# Autodesk Inventor assembly: fab model mk-1
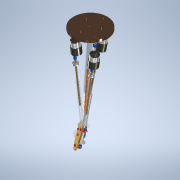
[picture p0: Inventor's stored thumbnail of the model, 180x180]
Saved by Autodesk Inventor 2020 (Build 240168000, 168)
## iProperties
Created: 2020-12-19
Part Number: fab model mk-1
Document SubType Name: Assembly
Designer: Vikki
Author: Vikki
## Documents named in this file (16)
- D:\borewell rescuebot\pll manipulator files\sps manipulator\fab model mk-1.iam
- D:\borewell rescuebot\pll manipulator files\sps manipulator\base.ipt
- D:\borewell rescuebot\pll manipulator files\sps manipulator\craftsman-3-pc-universal-joint-set-1.snapshot.1\Craftsman Socket U-Joint.iam
- D:\borewell rescuebot\pll manipulator files\sps manipulator\platform.ipt
- D:\borewell rescuebot\pll manipulator files\sps manipulator\JGB37-520.iam
- D:\borewell rescuebot\pll manipulator files\sps manipulator\leadscrew.ipt
- D:\borewell rescuebot\pll manipulator files\sps manipulator\coupler.ipt
- D:\borewell rescuebot\pll manipulator files\sps manipulator\telescopic boom1.ipt
- D:\borewell rescuebot\pll manipulator files\sps manipulator\boom 3.ipt
- D:\borewell rescuebot\pll manipulator files\sps manipulator\15.ipt
- D:\borewell rescuebot\pll manipulator files\sps manipulator\ball-pin.ipt
- D:\borewell rescuebot\2020 bot\borewell max sixe.ipt
- D:\borewell rescuebot\2020 bot\min size bore well.ipt
- D:\borewell rescuebot\pll manipulator files\sps manipulator\motor bracket.ipt
- D:\borewell rescuebot\pll manipulator files\sps manipulator\fab model mk-1\Design Accelerator\Bearing1.iam
- D:\borewell rescuebot\pll manipulator files\sps manipulator\connector plunger.ipt
## Components (39 placed, 15 different names)
1. base:1 — Mate:1, Mate:2, Mate:3, Mate:4, Mate:5, Mate:6, Angle:1, Mate:18, Mate:19, Flush:2, Angle:7, Mate:61, Flush:6
2. Craftsman Socket U-Joint:1 [sub-assembly] — Mate:1, Mate:2, Angle:2, Mate:25, Mate:34, Mate:35, Angle:9, Mate:69
3. Craftsman Socket U-Joint:2 [sub-assembly] — Mate:5, Mate:6, Angle:3, Mate:24, Mate:32, Mate:33, Angle:10, Mate:75
4. Craftsman Socket U-Joint:3 [sub-assembly] — Mate:3, Mate:4, Angle:1, Angle:2, Angle:3, Mate:23, Mate:29, Mate:30, Angle:8, Mate:72
5. platform:1 — Mate:7, Mate:8, Mate:9, Mate:10, Mate:11, Mate:12, Mate:16, Mate:17, Flush:2, Angle:6, Angle:7, Mate:63, Flush:8, Mate:64, Mate:65, Flush:9, Flush:10
6. Craftsman Socket U-Joint:4 [sub-assembly] — Mate:7, Mate:8, Mate:24, Mate:55, Mate:82, Mate:85
7. Craftsman Socket U-Joint:5 [sub-assembly] — Mate:9, Mate:12, Mate:25, Mate:53, Mate:86, Mate:88
8. Craftsman Socket U-Joint:6 [sub-assembly] — Mate:10, Mate:11, Mate:23, Mate:57, Mate:78, Mate:81
9. Craftsman Socket U-Joint:7 [sub-assembly] — Mate:16, Mate:17, Mate:26, Flush:1, Angle:6, Mate:52, Mate:60
10. Craftsman Socket U-Joint:8 [sub-assembly] — Mate:18, Mate:19, Angle:5, Mate:26, Flush:1, Mate:48, Mate:59
11. JGB37-520:1 [sub-assembly] — Mate:29, Mate:30, Angle:8, Mate:43, Mate:47, Mate:73, Mate:74
12. JGB37-520:2 [sub-assembly] — Mate:32, Mate:33, Angle:10, Mate:44, Mate:46, Mate:76, Mate:77
13. JGB37-520:3 [sub-assembly] — Mate:34, Mate:35, Angle:9, Mate:36, Mate:45, Flush:7, Mate:70
14. leadscrew:1 — Mate:36, Mate:37, Mate:38
15. coupler:1 — Mate:37, Mate:38, Mate:45, Mate:67
16. leadscrew:2
17. coupler:2 — Mate:43, Mate:47
18. leadscrew:3
19. coupler:3 — Mate:44, Mate:46
20. telescopic boom1:1 — Mate:48, Mate:51, Mate:59
21. boom 3:1 — Mate:51, Mate:52
22. 15:1 — Mate:53, Angle:13, Mate:87
23. 15:2 — Mate:57, Angle:12, Mate:79, Mate:80
24. 15:3 — Mate:55, Angle:11, Mate:83, Mate:84
25. ball-pin:1 — Mate:60
26. borewell max sixe:1 — Mate:61, Mate:62, Flush:5
27. min size bore well:1 — Mate:62, Flush:5, Flush:6
28. motor bracket:1 — Flush:7, Mate:66, Mate:69, Mate:70, Angle:13
29. Bearing:1 [sub-assembly] — Mate:63, Flush:8
30. Bearing:2 [sub-assembly] — Mate:64, Flush:10
31. Bearing:3 [sub-assembly] — Mate:65, Flush:9
32. Bearing:4 [sub-assembly] — Mate:66, Mate:67
33. motor bracket:2 — Flush:11, Mate:72, Mate:73, Mate:74, Angle:12
34. Bearing:5 [sub-assembly] — Flush:11
35. motor bracket:3 — Mate:75, Mate:76, Mate:77, Angle:11
36. Bearing:6 [sub-assembly]
37. connector plunger:1 — Mate:78, Mate:79, Mate:80, Mate:81
38. connector plunger:2 — Mate:86, Mate:87, Mate:88
39. connector plunger:3 — Mate:82, Mate:83, Mate:84, Mate:85
## Relationships (98: Mate 74, Angle 12, Flush 12)
- Mate:1: base:1 ↔ Craftsman Socket U-Joint:1
- Mate:2: base:1 ↔ Craftsman Socket U-Joint:1
- Mate:3: base:1 ↔ Craftsman Socket U-Joint:3
- Mate:4: base:1 ↔ Craftsman Socket U-Joint:3
- Mate:5: base:1 ↔ Craftsman Socket U-Joint:2
- Mate:6: base:1 ↔ Craftsman Socket U-Joint:2
- Mate:7: platform:1 ↔ Craftsman Socket U-Joint:4
- Mate:8: platform:1 ↔ Craftsman Socket U-Joint:4
- Mate:9: platform:1 ↔ Craftsman Socket U-Joint:5
- Mate:10: platform:1 ↔ Craftsman Socket U-Joint:6
- Mate:11: platform:1 ↔ Craftsman Socket U-Joint:6
- Mate:12: platform:1 ↔ Craftsman Socket U-Joint:5
- Angle:1 (30 deg): base:1 ↔ Craftsman Socket U-Joint:3
- Angle:2 (60 deg): Craftsman Socket U-Joint:1 ↔ Craftsman Socket U-Joint:3
- Angle:3 (120 deg): Craftsman Socket U-Joint:2 ↔ Craftsman Socket U-Joint:3
- Mate:16: platform:1 ↔ Craftsman Socket U-Joint:7
- Mate:17: platform:1 ↔ Craftsman Socket U-Joint:7
- Mate:18: base:1 ↔ Craftsman Socket U-Joint:8
- Mate:19: base:1 ↔ Craftsman Socket U-Joint:8
- Angle:5 (0 deg): Craftsman Socket U-Joint:8
- Mate:23: Craftsman Socket U-Joint:3 ↔ Craftsman Socket U-Joint:6
- Mate:24: Craftsman Socket U-Joint:2 ↔ Craftsman Socket U-Joint:4
- Mate:25: Craftsman Socket U-Joint:1 ↔ Craftsman Socket U-Joint:5
- Mate:26: Craftsman Socket U-Joint:7 ↔ Craftsman Socket U-Joint:8
- Flush:1: Craftsman Socket U-Joint:7 ↔ Craftsman Socket U-Joint:8
- Flush:2 (500 mm): base:1 ↔ platform:1
- Angle:6 (0 deg): platform:1 ↔ Craftsman Socket U-Joint:7
- Angle:7 (0 deg): base:1 ↔ platform:1
- Mate:29: Craftsman Socket U-Joint:3 ↔ JGB37-520:1
- Mate:30 (25 mm): Craftsman Socket U-Joint:3 ↔ JGB37-520:1
- Mate:32: Craftsman Socket U-Joint:2 ↔ JGB37-520:2
- Mate:33 (25 mm): Craftsman Socket U-Joint:2 ↔ JGB37-520:2
- Mate:34: Craftsman Socket U-Joint:1 ↔ JGB37-520:3
- Mate:35 (25 mm): Craftsman Socket U-Joint:1 ↔ JGB37-520:3
- Angle:8 (0 deg): Craftsman Socket U-Joint:3 ↔ JGB37-520:1
- Angle:9 (180 deg): Craftsman Socket U-Joint:1 ↔ JGB37-520:3
- Angle:10 (0 deg): Craftsman Socket U-Joint:2 ↔ JGB37-520:2
- Mate:36: JGB37-520:3 ↔ leadscrew:1
- Mate:37: leadscrew:1 ↔ coupler:1
- Mate:38 (-10 mm): leadscrew:1 ↔ coupler:1
- [Mate]: leadscrew:2 ↔ coupler:2
- [Mate] (-10 mm): leadscrew:2 ↔ coupler:2
- [Mate]: leadscrew:3 ↔ coupler:3
- [Mate] (-10 mm): leadscrew:3 ↔ coupler:3
- Mate:43: JGB37-520:1 ↔ coupler:2
- Mate:44: JGB37-520:2 ↔ coupler:3
- Mate:45 (5 mm): JGB37-520:3 ↔ coupler:1
- Mate:46 (5 mm): JGB37-520:2 ↔ coupler:3
- Mate:47 (5 mm): JGB37-520:1 ↔ coupler:2
- Mate:48: Craftsman Socket U-Joint:8 ↔ telescopic boom1:1
- Mate:51: telescopic boom1:1 ↔ boom 3:1
- Mate:52: Craftsman Socket U-Joint:7 ↔ boom 3:1
- Mate:53: Craftsman Socket U-Joint:5 ↔ 15:1
- Mate:55: Craftsman Socket U-Joint:4 ↔ 15:3
- Mate:57: Craftsman Socket U-Joint:6 ↔ 15:2
- Mate:59 (-5 mm): Craftsman Socket U-Joint:8 ↔ telescopic boom1:1
- Mate:60: Craftsman Socket U-Joint:7 ↔ ball-pin:1
- [Flush]: borewell max sixe:1 ↔ min size bore well:1
- [Flush]: borewell max sixe:1 ↔ min size bore well:1
- Mate:61: base:1 ↔ borewell max sixe:1
- Mate:62: borewell max sixe:1 ↔ min size bore well:1
- Flush:5: borewell max sixe:1 ↔ min size bore well:1
- Flush:6 (-400 mm): base:1 ↔ min size bore well:1
- Flush:7: JGB37-520:3 ↔ motor bracket:1
- Mate:63: platform:1 ↔ Bearing:1
- Flush:8: platform:1 ↔ Bearing:1
- Mate:64: platform:1 ↔ Bearing:2
- Mate:65: platform:1 ↔ Bearing:3
- Flush:9: platform:1 ↔ Bearing:3
- Flush:10: platform:1 ↔ Bearing:2
- Mate:66: motor bracket:1 ↔ Bearing:4
- Mate:67: coupler:1 ↔ Bearing:4
- [Mate]: motor bracket:2 ↔ Bearing:5
- Flush:11: motor bracket:2 ↔ Bearing:5
- Mate:69: Craftsman Socket U-Joint:1 ↔ motor bracket:1
- Mate:70: JGB37-520:3 ↔ motor bracket:1
- [Mate]: motor bracket:3 ↔ Bearing:6
- [Flush]: motor bracket:3 ↔ Bearing:6
- Mate:72: Craftsman Socket U-Joint:3 ↔ motor bracket:2
- Mate:73: JGB37-520:1 ↔ motor bracket:2
- Mate:74: JGB37-520:1 ↔ motor bracket:2
- Mate:75: Craftsman Socket U-Joint:2 ↔ motor bracket:3
- Mate:76: JGB37-520:2 ↔ motor bracket:3
- Mate:77: JGB37-520:2 ↔ motor bracket:3
- Angle:11 (180 deg): 15:3 ↔ motor bracket:3
- Angle:12 (180 deg): 15:2 ↔ motor bracket:2
- Angle:13 (180 deg): 15:1 ↔ motor bracket:1
- Mate:78: Craftsman Socket U-Joint:6 ↔ connector plunger:1
- Mate:79: 15:2 ↔ connector plunger:1
- Mate:80: 15:2 ↔ connector plunger:1
- Mate:81 (0.5 mm): Craftsman Socket U-Joint:6 ↔ connector plunger:1
- Mate:82: Craftsman Socket U-Joint:4 ↔ connector plunger:3
- Mate:83: 15:3 ↔ connector plunger:3
- Mate:84: 15:3 ↔ connector plunger:3
- Mate:85 (0.5 mm): Craftsman Socket U-Joint:4 ↔ connector plunger:3
- Mate:86: Craftsman Socket U-Joint:5 ↔ connector plunger:2
- Mate:87: 15:1 ↔ connector plunger:2
- Mate:88 (0.5 mm): Craftsman Socket U-Joint:5 ↔ connector plunger:2
## Named parameters: d70_d68 = 0 mm, d71_d69 = -10 mm, d72_d68 = 0 mm, d73_d69 = -10 mm, d121_d105 = 0 mm, d127_d124 = 0 mm, d128_d121_d105 = 0 mm
